# Autodesk Inventor assembly: Geneva drive
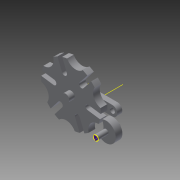
[picture p0: Inventor's stored thumbnail of the model, 180x180]
Saved by Autodesk Inventor 2018 (Build 220112000, 112)
## iProperties
Created: 2018-01-19
Part Number: Geneva drive
Document SubType Name: Assembly
Designer: Rus
Author: Rus
## Documents named in this file (4)
- E:\Libraries\3D Objects\Geneva drive\Mechanical\Attempt 1\Geneva drive Assembly.iam
- E:\Libraries\3D Objects\Geneva drive\Mechanical\Attempt 1\Geneva Drive.ipt
- E:\Libraries\3D Objects\Geneva drive\Mechanical\Attempt 1\Geneva Driven.ipt
- E:\Libraries\3D Objects\Geneva drive\Mechanical\Attempt 1\Frame.ipt
## Components (3 placed, 3 different names)
1. Geneva Drive:1
2. Geneva Driven:1 — Insert:1
3. Frame:1 — Insert:1
## Relationships (2: Mate 1, Insert 1)
- Mate:3 (87.9881 mm)
- Insert:1: Geneva Driven:1 ↔ Frame:1
